# Autodesk Inventor assembly: Structure
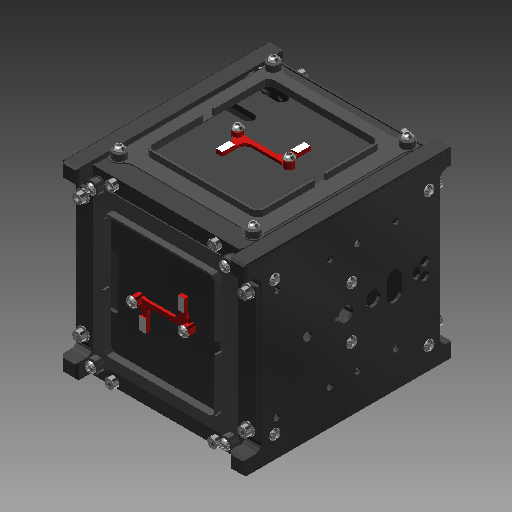
[picture p0: Inventor's stored thumbnail of the model, 512x512]
Saved by Autodesk Inventor 2018 (Build 220112000, 112)
## iProperties
Created: 2019-03-30
Part Number: Structure
Document SubType Name: Assembly
Designer: Bradley
Author: Bradley
## Documents named in this file (20)
- C:\Users\Bradley\Documents\GitHub\CougSat1-Hardware\CougSat1-Structure\CADModel\Imported\Structure.iam
- C:\Users\Bradley\Documents\GitHub\CougSat1-Hardware\CougSat1-Structure\CADModel\Imported\Structure_+X.ipt
- C:\Users\Bradley\Documents\GitHub\CougSat1-Hardware\CougSat1-Structure\CADModel\Imported\Structure_-X.ipt
- C:\Users\Bradley\Documents\GitHub\CougSat1-Hardware\CougSat1-Structure\CADModel\Imported\Structure_+Z.ipt
- C:\Users\Bradley\Documents\GitHub\CougSat1-Hardware\CougSat1-Structure\CADModel\Imported\Structure_Y.ipt
- C:\Users\Bradley\Documents\GitHub\CougSat1-Hardware\CougSat1-Structure\CADModel\Imported\Structure_-Z.ipt
- C:\Users\Bradley\Documents\GitHub\CougSat1-Hardware\CougSat1-Structure\CADModel\Imported\Structure_SolarPanelHeatsink.ipt
- C:\Users\Bradley\Documents\GitHub\CougSat1-Hardware\CougSat1-Structure\CADModel\Imported\Structure_MagnetorquerForm.ipt
- C:\Users\Bradley\Documents\GitHub\CougSat1-Hardware\CougSat1-Structure\CADModel\Imported\Structure_SwitchBlock.ipt
- C:\Users\Bradley\Documents\GitHub\CougSat1-Hardware\CougSat1-Structure\CADModel\Imported\Structure_SwitchPin.ipt
- C:\Users\Bradley\Documents\GitHub\Resources\SupplierDocuments\48 - Hardware\48-0360\48-0360.ipt
- C:\Users\Bradley\Documents\GitHub\Resources\SupplierDocuments\48 - Hardware\48-0361\48-0361.ipt
- C:\Users\Bradley\Documents\GitHub\Resources\SupplierDocuments\48 - Hardware\48-0340\48-0340.ipt
- C:\Users\Bradley\Documents\GitHub\Resources\SupplierDocuments\48 - Hardware\48-0380\48-0380.ipt
- C:\Users\Bradley\Documents\GitHub\Resources\SupplierDocuments\48 - Hardware\48-03A0\48-03A0.ipt
- C:\Users\Bradley\Documents\GitHub\Resources\SupplierDocuments\48 - Hardware\48-0350\48-0350.ipt
- C:\Users\Bradley\Documents\GitHub\Resources\SupplierDocuments\48 - Hardware\48-0150\48-0150.ipt
- C:\Users\Bradley\Documents\GitHub\Resources\SupplierDocuments\48 - Hardware\48-0300\48-0300.ipt
- C:\Users\Bradley\Documents\GitHub\Resources\SupplierDocuments\48 - Hardware\48-0001\48-0001.ipt
- C:\Users\Bradley\Documents\GitHub\Resources\SupplierDocuments\49 - Electromechanical\49-0001\49-0001.iam
## Components (83 placed, 19 different names)
1. 48-0001:1 — Insert:27
2. 48-0001:2 — Insert:28
3. 48-0150:1 — Insert:100
4. 48-0150:2 — Insert:99
5. 48-0300:1 — Insert:29, Insert:30
6. 48-0300:10 — Insert:42
7. 48-0300:11 — Insert:38
8. 48-0300:12 — Insert:54
9. 48-0300:2 — Insert:53
10. 48-0300:3 — Insert:51
11. 48-0300:4 — Insert:52
12. 48-0300:5 — Insert:83, Insert:87
13. 48-0300:6 — Insert:84, Insert:88
14. 48-0300:7 — Insert:85, Insert:90
15. 48-0300:8 — Insert:86, Insert:89
16. 48-0300:9 — Insert:41
17. 48-0340:1 — Insert:77
18. 48-0340:10 — Insert:90
19. 48-0340:2 — Insert:89
20. 48-0340:3 — Insert:78
21. 48-0340:4 — Insert:79
22. 48-0340:5 — Insert:80
23. 48-0340:6 — Insert:81
24. 48-0340:7 — Insert:82
25. 48-0340:8 — Insert:87
26. 48-0340:9 — Insert:88
27. 48-0350:1 — Insert:43
28. 48-0350:2 — Insert:44
29. 48-0350:3 — Insert:45
30. 48-0350:4 — Insert:46
31. 48-0350:5 — Insert:58
32. 48-0350:6 — Insert:57
33. 48-0350:7 — Insert:55
34. 48-0350:8 — Insert:56
35. 48-0360:1 — Insert:91
36. 48-0360:2 — Insert:92
37. 48-0360:3 — Insert:94
38. 48-0360:4 — Insert:93
39. 48-0361:1 — Insert:29
40. 48-0361:2
41. 48-0361:3
42. 48-0361:4
43. 48-0361:5
44. 48-0361:6
45. 48-0361:7
46. 48-0361:8
47. 48-0380:1 — Insert:59
48. 48-0380:10 — Insert:75
49. 48-0380:11 — Insert:60
50. 48-0380:12 — Insert:63
51. 48-0380:13 — Insert:64
52. 48-0380:14 — Insert:61
53. 48-0380:15 — Insert:62
54. 48-0380:16 — Insert:65
55. 48-0380:17 — Insert:66
56. 48-0380:18 — Insert:67
57. 48-0380:2 — Insert:68
58. 48-0380:3 — Insert:69
59. 48-0380:4 — Insert:70
60. 48-0380:5 — Insert:71
61. 48-0380:6 — Insert:72
62. 48-0380:7 — Insert:74
63. 48-0380:8 — Insert:73
64. 48-0380:9 — Insert:76
65. 48-03A0:1 — Insert:95
66. 48-03A0:2 — Insert:96
67. 49-0001:1 [sub-assembly] — Insert:97, Insert:98, Insert:99, Insert:100
68. Structure_+X:1 — Mate:1, Mate:2, Insert:1, Insert:2, Mate:3, Insert:9, Insert:10, Insert:27, Insert:77, Insert:78, Insert:79, Insert:80, Insert:81, Insert:82
69. Structure_+Z:1 — Insert:1, Insert:2, Insert:3, Insert:4, Insert:5, Insert:6, Insert:7, Insert:8, Insert:13, Insert:14, Insert:23, Insert:24, Insert:30, Insert:38, Insert:41, Insert:42, Insert:43, Insert:44, Insert:45, Insert:46
70. Structure_-X:1 — Insert:7, Insert:8, Insert:17, Insert:18, Insert:21, Insert:22, Insert:28, Insert:97, Insert:98, Insert:102, Angle:1
71. Structure_-Z:1 — Insert:9, Insert:10, Insert:51, Insert:52, Insert:53, Insert:54, Insert:55, Insert:56, Insert:57, Insert:58, Insert:83, Insert:84, Insert:85, Insert:86
72. Structure_MagnetorquerForm:1 — Insert:19, Insert:20, Insert:59, Insert:60, Insert:63, Insert:64
73. Structure_MagnetorquerForm:2 — Insert:21, Insert:22, Insert:91, Insert:92, Insert:93, Insert:94
74. Structure_MagnetorquerForm:3 — Insert:23, Insert:24, Insert:71, Insert:72, Insert:75, Insert:76
75. Structure_MagnetorquerForm:4 — Insert:25, Insert:26, Insert:65, Insert:66, Insert:69, Insert:70
76. Structure_SolarPanelHeatsink:1 — Insert:13, Insert:14, Insert:73, Insert:74
77. Structure_SolarPanelHeatsink:2 — Insert:11, Insert:12, Insert:61, Insert:62
78. Structure_SolarPanelHeatsink:3 — Insert:17, Insert:18, Insert:95, Insert:96
79. Structure_SolarPanelHeatsink:4 — Insert:15, Insert:16, Insert:67, Insert:68
80. Structure_SwitchBlock:1 — Insert:101, Angle:1
81. Structure_SwitchPin:1 — Insert:101, Insert:102
82. Structure_Y:1 — Insert:3, Insert:4, Insert:11, Insert:12, Insert:19, Insert:20
83. Structure_Y:2 — Insert:5, Insert:6, Insert:15, Insert:16, Insert:25, Insert:26
## Relationships (100: Insert 96, Mate 3, Angle 1)
- Mate:1 (50 mm): Structure_+X:1
- Mate:2 (-49 mm): Structure_+X:1
- Insert:1: Structure_+X:1 ↔ Structure_+Z:1
- Insert:2: Structure_+X:1 ↔ Structure_+Z:1
- Insert:3: Structure_+Z:1 ↔ Structure_Y:1
- Insert:4: Structure_+Z:1 ↔ Structure_Y:1
- Insert:5: Structure_+Z:1 ↔ Structure_Y:2
- Insert:6: Structure_+Z:1 ↔ Structure_Y:2
- Insert:7: Structure_+Z:1 ↔ Structure_-X:1
- Insert:8: Structure_+Z:1 ↔ Structure_-X:1
- Mate:3 (50 mm): Structure_+X:1
- Insert:9: Structure_+X:1 ↔ Structure_-Z:1
- Insert:10: Structure_+X:1 ↔ Structure_-Z:1
- Insert:11: Structure_SolarPanelHeatsink:2 ↔ Structure_Y:1
- Insert:12: Structure_SolarPanelHeatsink:2 ↔ Structure_Y:1
- Insert:13: Structure_+Z:1 ↔ Structure_SolarPanelHeatsink:1
- Insert:14: Structure_+Z:1 ↔ Structure_SolarPanelHeatsink:1
- Insert:15: Structure_SolarPanelHeatsink:4 ↔ Structure_Y:2
- Insert:16: Structure_SolarPanelHeatsink:4 ↔ Structure_Y:2
- Insert:17: Structure_-X:1 ↔ Structure_SolarPanelHeatsink:3
- Insert:18: Structure_-X:1 ↔ Structure_SolarPanelHeatsink:3
- Insert:19: Structure_MagnetorquerForm:1 ↔ Structure_Y:1
- Insert:20: Structure_MagnetorquerForm:1 ↔ Structure_Y:1
- Insert:21: Structure_-X:1 ↔ Structure_MagnetorquerForm:2
- Insert:22: Structure_-X:1 ↔ Structure_MagnetorquerForm:2
- Insert:23: Structure_+Z:1 ↔ Structure_MagnetorquerForm:3
- Insert:24: Structure_+Z:1 ↔ Structure_MagnetorquerForm:3
- Insert:25: Structure_MagnetorquerForm:4 ↔ Structure_Y:2
- Insert:26: Structure_MagnetorquerForm:4 ↔ Structure_Y:2
- Insert:27: 48-0001:1 ↔ Structure_+X:1
- Insert:28: 48-0001:2 ↔ Structure_-X:1
- Insert:29: 48-0300:1 ↔ 48-0361:1
- Insert:30: 48-0300:1 ↔ Structure_+Z:1
- [Insert]: 48-0300:9 ↔ 48-0361:5
- [Insert]: 48-0300:10 ↔ 48-0361:6
- [Insert]: 48-0300:11 ↔ 48-0361:7
- Insert:38: 48-0300:11 ↔ Structure_+Z:1
- Insert:41: 48-0300:9 ↔ Structure_+Z:1
- Insert:42: 48-0300:10 ↔ Structure_+Z:1
- Insert:43: 48-0350:1 ↔ Structure_+Z:1
- Insert:44: 48-0350:2 ↔ Structure_+Z:1
- Insert:45: 48-0350:3 ↔ Structure_+Z:1
- Insert:46: 48-0350:4 ↔ Structure_+Z:1
- [Insert]: 48-0300:12 ↔ 48-0361:8
- [Insert]: 48-0300:2 ↔ 48-0361:2
- [Insert]: 48-0300:3 ↔ 48-0361:3
- [Insert]: 48-0300:4 ↔ 48-0361:4
- Insert:51: 48-0300:3 ↔ Structure_-Z:1
- Insert:52: 48-0300:4 ↔ Structure_-Z:1
- Insert:53: 48-0300:2 ↔ Structure_-Z:1
- Insert:54: 48-0300:12 ↔ Structure_-Z:1
- Insert:55: 48-0350:7 ↔ Structure_-Z:1
- Insert:56: 48-0350:8 ↔ Structure_-Z:1
- Insert:57: 48-0350:6 ↔ Structure_-Z:1
- Insert:58: 48-0350:5 ↔ Structure_-Z:1
- Insert:59 (0.6 mm): 48-0380:1 ↔ Structure_MagnetorquerForm:1
- Insert:60 (0.6 mm): 48-0380:11 ↔ Structure_MagnetorquerForm:1
- Insert:61 (0.6 mm): 48-0380:14 ↔ Structure_SolarPanelHeatsink:2
- Insert:62 (0.6 mm): 48-0380:15 ↔ Structure_SolarPanelHeatsink:2
- Insert:63 (0.6 mm): 48-0380:12 ↔ Structure_MagnetorquerForm:1
- Insert:64 (0.6 mm): 48-0380:13 ↔ Structure_MagnetorquerForm:1
- Insert:65 (0.6 mm): 48-0380:16 ↔ Structure_MagnetorquerForm:4
- Insert:66 (0.6 mm): 48-0380:17 ↔ Structure_MagnetorquerForm:4
- Insert:67 (0.6 mm): 48-0380:18 ↔ Structure_SolarPanelHeatsink:4
- Insert:68 (0.6 mm): 48-0380:2 ↔ Structure_SolarPanelHeatsink:4
- Insert:69 (0.6 mm): 48-0380:3 ↔ Structure_MagnetorquerForm:4
- Insert:70 (0.6 mm): 48-0380:4 ↔ Structure_MagnetorquerForm:4
- Insert:71 (0.6 mm): 48-0380:5 ↔ Structure_MagnetorquerForm:3
- Insert:72 (0.6 mm): 48-0380:6 ↔ Structure_MagnetorquerForm:3
- Insert:73 (0.6 mm): 48-0380:8 ↔ Structure_SolarPanelHeatsink:1
- Insert:74 (0.6 mm): 48-0380:7 ↔ Structure_SolarPanelHeatsink:1
- Insert:75 (0.6 mm): 48-0380:10 ↔ Structure_MagnetorquerForm:3
- Insert:76 (0.6 mm): 48-0380:9 ↔ Structure_MagnetorquerForm:3
- Insert:77 (0.6 mm): 48-0340:1 ↔ Structure_+X:1
- Insert:78 (0.6 mm): 48-0340:3 ↔ Structure_+X:1
- Insert:79 (0.6 mm): 48-0340:4 ↔ Structure_+X:1
- Insert:80 (0.6 mm): 48-0340:5 ↔ Structure_+X:1
- Insert:81 (0.6 mm): 48-0340:6 ↔ Structure_+X:1
- Insert:82 (0.6 mm): 48-0340:7 ↔ Structure_+X:1
- Insert:83: 48-0300:5 ↔ Structure_-Z:1
- Insert:84: 48-0300:6 ↔ Structure_-Z:1
- Insert:85: 48-0300:7 ↔ Structure_-Z:1
- Insert:86: 48-0300:8 ↔ Structure_-Z:1
- Insert:87 (0.6 mm): 48-0300:5 ↔ 48-0340:8
- Insert:88 (0.6 mm): 48-0300:6 ↔ 48-0340:9
- Insert:89 (0.6 mm): 48-0300:8 ↔ 48-0340:2
- Insert:90 (0.6 mm): 48-0300:7 ↔ 48-0340:10
- Insert:91 (0.6 mm): 48-0360:1 ↔ Structure_MagnetorquerForm:2
- Insert:92 (0.6 mm): 48-0360:2 ↔ Structure_MagnetorquerForm:2
- Insert:93 (0.6 mm): 48-0360:4 ↔ Structure_MagnetorquerForm:2
- Insert:94 (0.6 mm): 48-0360:3 ↔ Structure_MagnetorquerForm:2
- Insert:95 (0.6 mm): 48-03A0:1 ↔ Structure_SolarPanelHeatsink:3
- Insert:96 (0.6 mm): 48-03A0:2 ↔ Structure_SolarPanelHeatsink:3
- Insert:97: 49-0001:1 ↔ Structure_-X:1
- Insert:98: 49-0001:1 ↔ Structure_-X:1
- Insert:99: 48-0150:2 ↔ 49-0001:1
- Insert:100: 48-0150:1 ↔ 49-0001:1
- Insert:101: Structure_SwitchBlock:1 ↔ Structure_SwitchPin:1
- Insert:102 (-0.75 mm): Structure_-X:1 ↔ Structure_SwitchPin:1
- Angle:1 (0 deg): Structure_-X:1 ↔ Structure_SwitchBlock:1
## Named parameters: d36_d32 = 0 mm, d37_d32 = 0 mm, d40_d32 = 0 mm, d52_d32 = 0 mm, d53_d32 = 0 mm, d54_d32 = 0 mm, d55_d32 = 0 mm, SolarPanelThickness = 0.6 mm, PXThickness = 0.6 mm, NZThickness = 0.6 mm
